# Autodesk Inventor assembly: Peep
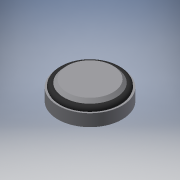
[picture p0: Inventor's stored thumbnail of the model, 180x180]
Saved by Autodesk Inventor 2018 (Build 220112000, 112)
## iProperties
Created: 2020-03-27
Part Number: Peep
Document SubType Name: Assembly
Designer: emile
Author: emile
## Documents named in this file (3)
- C:\Users\emile\OneDrive\Documents\Inventor\Respirator\Peep\Peep.iam
- C:\Users\emile\OneDrive\Documents\Inventor\Respirator\Peep\Diaphragme.ipt
- C:\Users\emile\OneDrive\Documents\Inventor\Respirator\Peep\9555K330_FOOD-AND-BEVERAGE O-RING.ipt
## Components (2 placed, 2 different names)
1. Diaphragme:1 — Mate:1, Tangent:1
2. 9555K330_FOOD-AND-BEVERAGE O-RING:1 — Mate:1, Tangent:1
## Relationships (2: Mate 1, Tangent 1)
- Mate:1: Diaphragme:1 ↔ 9555K330_FOOD-AND-BEVERAGE O-RING:1
- Tangent:1: Diaphragme:1 ↔ 9555K330_FOOD-AND-BEVERAGE O-RING:1
